# Autodesk Inventor assembly: TOF Assembly
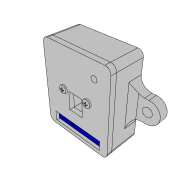
[picture p0: Inventor's stored thumbnail of the model, 180x180]
Saved by Autodesk Inventor 2019.3 (Build 233278000, 278)
## iProperties
Created: 2019-02-11
Part Number: TOF Assembly
Document SubType Name: Assembly
Designer: erics
Mass: 26.1245 g
Surface Area: 249.209 cm^2
Volume: 24.9346 cm^3
Density: 1.04772 g/cm^3
Author: erics
## Documents named in this file (6)
- D:\Users\erics\Documents\ToF-CAN\hardware\CAD\TOF Assembly.iam
- D:\Users\erics\Documents\ToF-CAN\hardware\CAD\CAN TOF\CAN TOF.iam
- D:\Users\erics\Documents\CAD Library\Electronics\Adafruit VL53L0X.ipt
- D:\Users\erics\Documents\ToF-CAN\hardware\CAD\TOF Case P1.ipt
- D:\Users\erics\Documents\ToF-CAN\hardware\CAD\TOF Case P2_ISO.ipt
- D:\Users\erics\Documents\Inventor\Content Center Files\R2019\en-US\ANSI B18.6.3(03)\ANSI B18.6.3 - 2-56 UNC - 0.75(14).ipt
## Components (6 placed, 5 different names)
1. CAN TOF:1 [sub-assembly] — Mate:1, Mate:2, Mate:3, Mate:4, Mate:5, Mate:6
2. Adafruit VL53L0X:1 — Mate:1, Mate:2, Mate:3
3. TOF Case P1:1 — Mate:4, Mate:5, Mate:6, Flush:1, Flush:2, Mate:7
4. TOF Case P2_ISO:1 — Flush:1, Flush:2, Mate:7, Insert:1, Insert:2
5. Cross Recessed Binding Head Machine Screw - Type I - Inch No. 2 - 56 - 3/4:1 — Insert:2
6. Cross Recessed Binding Head Machine Screw - Type I - Inch No. 2 - 56 - 3/4:2 — Insert:1
## Relationships (11: Mate 7, Flush 2, Insert 2)
- Mate:1: CAN TOF:1 ↔ Adafruit VL53L0X:1
- Mate:2: CAN TOF:1 ↔ Adafruit VL53L0X:1
- Mate:3: CAN TOF:1 ↔ Adafruit VL53L0X:1
- Mate:4: CAN TOF:1 ↔ TOF Case P1:1
- Mate:5: CAN TOF:1 ↔ TOF Case P1:1
- Mate:6: CAN TOF:1 ↔ TOF Case P1:1
- Flush:1: TOF Case P1:1 ↔ TOF Case P2_ISO:1
- Flush:2: TOF Case P1:1 ↔ TOF Case P2_ISO:1
- Mate:7: TOF Case P1:1 ↔ TOF Case P2_ISO:1
- Insert:1: TOF Case P2_ISO:1 ↔ Cross Recessed Binding Head Machine Screw - Type I - Inch No. 2 - 56 - 3/4:2
- Insert:2: TOF Case P2_ISO:1 ↔ Cross Recessed Binding Head Machine Screw - Type I - Inch No. 2 - 56 - 3/4:1
